# Autodesk Inventor assembly: DriveTrain
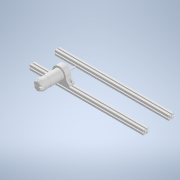
[picture p0: Inventor's stored thumbnail of the model, 180x180]
Saved by Autodesk Inventor 2020 (Build 240168000, 168)
## iProperties
Created: 2020-01-29
Part Number: DriveTrain
Document SubType Name: Assembly
Designer: yukin
Author: yukin
## Documents named in this file (4)
- C:\Users\yukin\OneDrive\Desktop\DriveTrain.iam
- C:\Users\yukin\Downloads\1inchExtrusion.ipt
- C:\Users\yukin\Downloads\REV-41-1298 (1).iam
- C:\Users\yukin\Downloads\Motor_Mount_vCAD.ipt
## Components (4 placed, 3 different names)
1. 1inchExtrusion:1 — Flush:1, Flush:2, Tangent:1, Flush:3, Flush:4, Tangent:2, Flush:5, Mate:2
2. 1inchExtrusion:2 — Flush:1, Flush:2
3. REV-41-1298 (1):1 [sub-assembly] — Tangent:1, Flush:3, Flush:4, Tangent:2, Rotational:1
4. Motor_Mount_vCAD:1 — Flush:5, Mate:2, Rotational:1
## Relationships (9: Flush 5, Tangent 2, Mate 1, RevoluteJoint 1)
- Flush:1: 1inchExtrusion:1 ↔ 1inchExtrusion:2
- Flush:2: 1inchExtrusion:1 ↔ 1inchExtrusion:2
- Tangent:1: 1inchExtrusion:1 ↔ REV-41-1298 (1):1
- Flush:3: 1inchExtrusion:1 ↔ REV-41-1298 (1):1
- Flush:4: 1inchExtrusion:1 ↔ REV-41-1298 (1):1
- Tangent:2: 1inchExtrusion:1 ↔ REV-41-1298 (1):1
- Flush:5: 1inchExtrusion:1 ↔ Motor_Mount_vCAD:1
- Mate:2: 1inchExtrusion:1 ↔ Motor_Mount_vCAD:1
- Rotational:1 [RevoluteJoint]: REV-41-1298 (1):1 ↔ Motor_Mount_vCAD:1
